# Autodesk Inventor assembly: bed_assembly
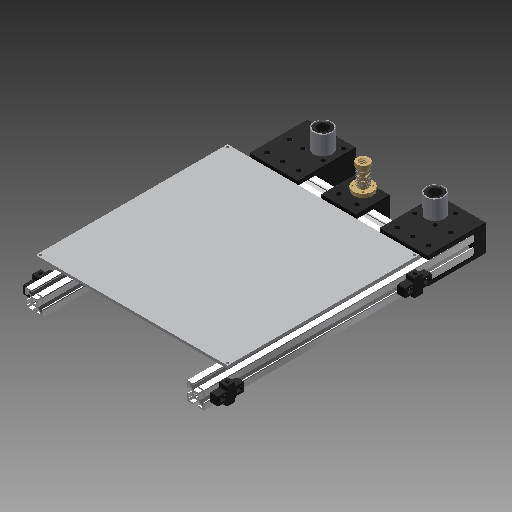
[picture p0: Inventor's stored thumbnail of the model, 512x512]
Saved by Autodesk Inventor 2018 (Build 220112000, 112)
## iProperties
Created: 2018-05-24
Part Number: bed_assembly
Document SubType Name: Assembly
Designer: Z. Deniz
Author: Z. Deniz
## Documents named in this file (10)
- C:\Users\zdeni\Desktop\my3D\3D_Model_v2\montajlar\bed_assembly.iam
- C:\Users\zdeni\Desktop\my3D\3D_Model_v2\parçalar\2020 Extrusion 160mm.ipt
- C:\Users\zdeni\Desktop\my3D\3D_Model_v2\parçalar\bed_pulley_holder.ipt
- C:\Users\zdeni\Desktop\my3D\3D_Model_v2\parçalar\90 angle.ipt
- C:\Users\zdeni\Desktop\my3D\3D_Model_v2\parçalar\modeller\HEATBED MK3.ipt
- C:\Users\zdeni\Desktop\my3D\3D_Model_v2\parçalar\modeller\123LMK12LUU.ipt
- C:\Users\zdeni\Desktop\my3D\3D_Model_v2\parçalar\z_nut_holder.ipt
- C:\Users\zdeni\Desktop\my3D\3D_Model_v2\parçalar\modeller\123TR8_8(P4) Antibacklash Nut w. spring.ipt
- C:\Users\zdeni\Desktop\my3D\3D_Model_v2\parçalar\2020 Extrusion 300mm.ipt
- C:\Users\zdeni\Desktop\my3D\3D_Model_v2\parçalar\bed_spring_holder_v3.ipt
## Components (16 placed, 9 different names)
1. 2020 Extrusion 160mm:1 — Mate:3, Mate:6, Mate:8, Mate:9, Mate:11, Mate:30, Mate:31, Mate:39, Flush:1, Flush:2, Flush:3, Flush:5, Mate:55
2. bed_pulley_holder:1 — Mate:8, Mate:9, Tangent:2, Mate:17, Tangent:7, Mate:32, Flush:1, Mate:41
3. 90 angle:1 — Mate:6, Mate:40, Flush:4
4. 90 angle:2 — Mate:3, Flush:2, Flush:3, Mate:42
5. bed_pulley_holder:2 — Mate:11, Mate:13, Tangent:1, Mate:16, Tangent:6, Mate:36, Mate:37, Mate:38
6. HEATBED MK3:1 — Mate:47, Mate:48, Mate:49, Mate:50, Mate:51, Mate:52, Mate:53, Mate:54, Mate:55
7. 123LMK12LUU:1 — Tangent:1, Mate:16, Tangent:6
8. 123LMK12LUU:2 — Tangent:2, Mate:17, Tangent:7
9. z_nut_holder:1 — Mate:30, Mate:31, Mate:32, Mate:33, Mate:34, Mate:35
10. 123TR8_8(P4) Antibacklash Nut w. spring:1 — Mate:33, Mate:34, Mate:35
11. 2020 Extrusion 300mm:1 — Mate:36, Mate:37, Mate:38, Mate:39, Mate:40, Flush:4, Mate:45, Mate:46
12. 2020 Extrusion 300mm:2 — Mate:41, Mate:42, Flush:5, Mate:43, Mate:44, Flush:6
13. bed_spring_holder_v3:1 — Mate:43, Mate:47, Mate:49, Flush:6
14. bed_spring_holder_v3:2 — Mate:44, Mate:48, Mate:50
15. bed_spring_holder_v3:3 — Mate:45, Mate:53, Mate:54
16. bed_spring_holder_v3:4 — Mate:46, Mate:51, Mate:52
## Relationships (44: Mate 34, Flush 6, Tangent 4)
- Mate:3: 2020 Extrusion 160mm:1 ↔ 90 angle:2
- Mate:6: 2020 Extrusion 160mm:1 ↔ 90 angle:1
- Mate:8: 2020 Extrusion 160mm:1 ↔ bed_pulley_holder:1
- Mate:9: 2020 Extrusion 160mm:1 ↔ bed_pulley_holder:1
- Mate:11: 2020 Extrusion 160mm:1 ↔ bed_pulley_holder:2
- Mate:13: bed_pulley_holder:2
- Tangent:1: bed_pulley_holder:2 ↔ 123LMK12LUU:1
- Mate:16: bed_pulley_holder:2 ↔ 123LMK12LUU:1
- Tangent:2: bed_pulley_holder:1 ↔ 123LMK12LUU:2
- Mate:17: bed_pulley_holder:1 ↔ 123LMK12LUU:2
- Tangent:6: bed_pulley_holder:2 ↔ 123LMK12LUU:1
- Tangent:7: bed_pulley_holder:1 ↔ 123LMK12LUU:2
- Mate:30: 2020 Extrusion 160mm:1 ↔ z_nut_holder:1
- Mate:31: 2020 Extrusion 160mm:1 ↔ z_nut_holder:1
- Mate:32 (25 mm): bed_pulley_holder:1 ↔ z_nut_holder:1
- Mate:33: z_nut_holder:1 ↔ 123TR8_8(P4) Antibacklash Nut w. spring:1
- Mate:34: z_nut_holder:1 ↔ 123TR8_8(P4) Antibacklash Nut w. spring:1
- Mate:35: z_nut_holder:1 ↔ 123TR8_8(P4) Antibacklash Nut w. spring:1
- Mate:36: bed_pulley_holder:2 ↔ 2020 Extrusion 300mm:1
- Mate:37: bed_pulley_holder:2 ↔ 2020 Extrusion 300mm:1
- Mate:38: bed_pulley_holder:2 ↔ 2020 Extrusion 300mm:1
- Mate:39: 2020 Extrusion 160mm:1 ↔ 2020 Extrusion 300mm:1
- Flush:1: 2020 Extrusion 160mm:1 ↔ bed_pulley_holder:1
- Flush:2: 2020 Extrusion 160mm:1 ↔ 90 angle:2
- Flush:3 (1.5 mm): 2020 Extrusion 160mm:1 ↔ 90 angle:2
- Mate:40: 90 angle:1 ↔ 2020 Extrusion 300mm:1
- Flush:4 (1.5 mm): 90 angle:1 ↔ 2020 Extrusion 300mm:1
- Mate:41: bed_pulley_holder:1 ↔ 2020 Extrusion 300mm:2
- Mate:42: 90 angle:2 ↔ 2020 Extrusion 300mm:2
- Flush:5: 2020 Extrusion 160mm:1 ↔ 2020 Extrusion 300mm:2
- Mate:43: 2020 Extrusion 300mm:2 ↔ bed_spring_holder_v3:1
- Mate:44: 2020 Extrusion 300mm:2 ↔ bed_spring_holder_v3:2
- Mate:45: 2020 Extrusion 300mm:1 ↔ bed_spring_holder_v3:3
- Mate:46: 2020 Extrusion 300mm:1 ↔ bed_spring_holder_v3:4
- Mate:47: HEATBED MK3:1 ↔ bed_spring_holder_v3:1
- Mate:48: HEATBED MK3:1 ↔ bed_spring_holder_v3:2
- Mate:49 (15 mm): HEATBED MK3:1 ↔ bed_spring_holder_v3:1
- Mate:50 (15 mm): HEATBED MK3:1 ↔ bed_spring_holder_v3:2
- Flush:6: 2020 Extrusion 300mm:2 ↔ bed_spring_holder_v3:1
- Mate:51 (15 mm): HEATBED MK3:1 ↔ bed_spring_holder_v3:4
- Mate:52: HEATBED MK3:1 ↔ bed_spring_holder_v3:4
- Mate:53: HEATBED MK3:1 ↔ bed_spring_holder_v3:3
- Mate:54 (15 mm): HEATBED MK3:1 ↔ bed_spring_holder_v3:3
- Mate:55 (17 mm): 2020 Extrusion 160mm:1 ↔ HEATBED MK3:1
## Named parameters: back_space = 17.5 mm, spring_height = 15 mm
